# Autodesk Inventor assembly: s-assy-gripper
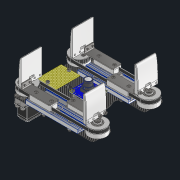
[picture p0: Inventor's stored thumbnail of the model, 180x180]
Saved by Autodesk Inventor 2021 (Build 250183000, 183)
## iProperties
Created: 2021-08-06
Part Number: s-assy-gripper
Document SubType Name: Assembly
Designer: yuta0
Mass: 588.108 g
Surface Area: 2137.5 cm^2
Volume: 253.038 cm^3
Density: 2.32419 g/cm^3
Author: yuta0
## Documents named in this file (25)
- C:\Users\yuta0\Documents\GitHub\catchrobo_hardware\assy-robot\s-assy-gripper.iam
- C:\Users\yuta0\Documents\GitHub\catchrobo_hardware\assy-robot\carbon_plate14.ipt
- C:\Users\yuta0\Documents\GitHub\catchrobo_hardware\assy-robot\mrs20-100.ipt
- C:\Users\yuta0\Documents\GitHub\catchrobo_hardware\assy-robot\mr-20cs_1.iam
- C:\Users\yuta0\Documents\GitHub\catchrobo_hardware\assy-robot\belt4.ipt
- C:\Users\yuta0\Documents\GitHub\catchrobo_hardware\assy-robot\base37.ipt
- C:\Users\yuta0\Documents\GitHub\catchrobo_hardware\assy-robot\USB Cam model ELP-USBFHD01M-L21.ipt
- C:\Users\yuta0\Documents\GitHub\catchrobo_hardware\assy-robot\CB3-5.ipt
- C:\Users\yuta0\Documents\GitHub\catchrobo_hardware\assy-robot\base38.ipt
- C:\Users\yuta0\Documents\GitHub\catchrobo_hardware\assy-robot\CB3-30.ipt
- C:\Users\yuta0\Documents\GitHub\catchrobo_hardware\assy-robot\LBNR4.ipt
- C:\Users\yuta0\Documents\GitHub\catchrobo_hardware\assy-robot\ARU-2010.ipt
- C:\Users\yuta0\Documents\GitHub\catchrobo_hardware\assy-robot\CB2-4.ipt
- C:\Users\yuta0\Documents\GitHub\catchrobo_hardware\assy-robot\d_type_board.ipt
- C:\Users\yuta0\Documents\GitHub\catchrobo_hardware\assy-robot\hexagonal_spacer_M3_5mm.ipt
- C:\Users\yuta0\Documents\GitHub\catchrobo_hardware\assy-robot\LBNR3.ipt
- C:\Users\yuta0\Documents\GitHub\catchrobo_hardware\assy-robot\steel_plate1.ipt
- C:\Users\yuta0\Documents\GitHub\catchrobo_hardware\assy-robot\CBSTNR3-16.ipt
- C:\Users\yuta0\Documents\GitHub\catchrobo_hardware\assy-robot\s-assy-rc_servo.iam
- C:\Users\yuta0\Documents\GitHub\catchrobo_hardware\assy-robot\s-assy-gripper_tentioner.iam
- C:\Users\yuta0\Documents\GitHub\catchrobo_hardware\assy-robot\FU650AD5-C6.ipt
- C:\Users\yuta0\Documents\GitHub\catchrobo_hardware\assy-robot\base21.ipt
- C:\Users\yuta0\Documents\GitHub\catchrobo_hardware\assy-robot\CBSTSR4-14.ipt
- C:\Users\yuta0\Documents\GitHub\catchrobo_hardware\assy-robot\base22.ipt
- C:\Users\yuta0\Documents\GitHub\catchrobo_hardware\assy-robot\CB3-10.ipt
## Components (93 placed, 24 different names)
1. carbon_plate14:1 — メイト:1, メイト:2, メイト:3, メイト:51, メイト:52, メイト:53, メイト:88, メイト:89, メイト:90, メイト:92, 角度:1, メイト:98, メイト:102, メイト:103, メイト:104, メイト:105, メイト:106, メイト:107, メイト:109, メイト:110, メイト:111, メイト:113, メイト:139, メイト:140, メイト:141, メイト:142, メイト:143, メイト:144, メイト:147, メイト:148, メイト:150, メイト:151, メイト:183, メイト:197, メイト:200, 角度:4, 角度:5, メイト:201, メイト:202, メイト:203, メイト:207, メイト:208
2. s-assy-rc_servo:1 [sub-assembly] — メイト:139, メイト:140, メイト:141, メイト:145, メイト:146
3. s-assy-rc_servo:2 [sub-assembly] — メイト:142, メイト:143, メイト:144, メイト:153, メイト:154
4. s-assy-gripper_tentioner:1 [sub-assembly] — メイト:147, メイト:148, メイト:149
5. s-assy-gripper_tentioner:2 [sub-assembly] — メイト:150, メイト:151, メイト:152
6. USB Cam model ELP-USBFHD01M-L21:1 — メイト:51, メイト:52, メイト:53, メイト:99, メイト:100, メイト:101
7. hexagonal_spacer_M3_5mm:1 — メイト:106, メイト:107, メイト:108, メイト:114
8. LBNR3:1 — メイト:108, メイト:109
9. LBNR3:2 — メイト:112, メイト:113
10. hexagonal_spacer_M3_5mm:2 — メイト:110, メイト:111, メイト:112
11. d_type_board:1 — メイト:104, メイト:105, メイト:114, メイト:115, メイト:116, メイト:117, メイト:118
12. CB3-5:11 — メイト:115, メイト:116
13. CB3-5:12 — メイト:117, メイト:118
14. belt4:1 — メイト:145, メイト:146, メイト:149
15. belt4:2 — メイト:152, メイト:153, メイト:154
16. FU650AD5-C6:1 — メイト:197, メイト:198, 角度:5
17. FU650AD5-C6:2 — メイト:199, メイト:200, 角度:4
18. base21:1 — メイト:201, メイト:202, メイト:203, メイト:204, メイト:205
19. base21:2 — メイト:206, メイト:207, メイト:208, メイト:209, メイト:210
20. CB3-30:1 — メイト:88, メイト:89
21. CB3-30:2
22. CB3-30:3
23. CB3-30:4
24. CB3-30:5
25. CB3-30:6
26. ARU-2010:1 — メイト:98, メイト:99
27. CB2-4:1 — メイト:100, メイト:101
28. CB2-4:2 — メイト:102, メイト:103
29. ARU-2010:2
30. CB2-4:3
31. CB2-4:6
32. ARU-2010:3
33. CB2-4:4
34. CB2-4:7
35. ARU-2010:4
36. CB2-4:5
37. CB2-4:8
38. CBSTNR3-16:4 — メイト:194, メイト:211
39. CBSTNR3-16:3 — メイト:193
40. steel_plate1:2 — メイト:195, メイト:196, メイト:212, メイト:213, メイト:214
41. base38:2 — メイト:195, メイト:196
42. base37:2 — メイト:211
43. mr-20cs_1:2 [sub-assembly] — メイト:193, メイト:194
44. CBSTSR4-14:1
45. LBNR4:4 — メイト:204
46. CBSTSR4-14:2
47. LBNR4:3 — メイト:205
48. base22:1 — メイト:212, メイト:213, メイト:214, メイト:215, メイト:216, メイト:217, メイト:218
49. CB3-10:1 — メイト:215, メイト:216
50. CB3-10:2 — メイト:217, メイト:218
51. mrs20-100:2 — メイト:183, メイト:198
52. CBSTNR3-16:5
53. CBSTNR3-16:6
54. steel_plate1:3
55. base38:3
56. base37:3
57. mr-20cs_1:3 [sub-assembly]
58. CBSTSR4-14:5
59. LBNR4:5
60. CBSTSR4-14:6
61. LBNR4:6
62. base22:3
63. CB3-10:5
64. CB3-10:6
65. mrs20-100:3
66. steel_plate1:1 — メイト:129, メイト:130, メイト:131, メイト:133, メイト:134, メイト:135, メイト:219, メイト:220, メイト:221
67. CBSTNR3-16:1 — メイト:132, メイト:133
68. CBSTNR3-16:2 — メイト:134, メイト:135
69. base37:1 — メイト:45, メイト:46, メイト:47, メイト:70, メイト:71, メイト:72
70. base38:1 — メイト:70, メイト:71, メイト:72, メイト:129, メイト:130, メイト:131, メイト:132
71. mr-20cs_1:1 [sub-assembly] — メイト:7, メイト:8, フラッシュ:1, メイト:45, メイト:46, メイト:47
72. mrs20-100:1 — フラッシュ:1, メイト:1, メイト:2, メイト:3, メイト:7, メイト:8, メイト:199
73. CBSTSR4-14:3
74. LBNR4:1 — メイト:90, 角度:2, メイト:210
75. CBSTSR4-14:4 — メイト:206
76. LBNR4:2 — メイト:92, 角度:1, 角度:2, メイト:209
77. CB3-10:4 — メイト:223
78. CB3-10:3 — メイト:222
79. base22:2 — メイト:219, メイト:220, メイト:221, メイト:222, メイト:223
80. steel_plate1:4
81. CBSTNR3-16:7
82. CBSTNR3-16:8
83. base37:4
84. base38:4
85. mr-20cs_1:4 [sub-assembly]
86. mrs20-100:4
87. CBSTSR4-14:7
88. LBNR4:7
89. CBSTSR4-14:8
90. LBNR4:8
91. CB3-10:7
92. CB3-10:8
93. base22:4
## Component patterns: (6 elements, first: CB3-30:1), (4 elements, first: ARU-2010:1 + CB2-4:1 + CB2-4:2), (2 elements, first: CBSTNR3-16:4 + CBSTNR3-16:3 + steel_plate1:2 + base38:2 + base37:2 + mr-20cs_1:2 + CBSTSR4-14:1 + LBNR4:4 + CBSTSR4-14:2 + LBNR4:3 + base22:1 + CB3-10:1 + CB3-10:2 + mrs20-100:2), (2 elements, first: steel_plate1:1 + CBSTNR3-16:1 + CBSTNR3-16:2 + base37:1 + base38:1 + mr-20cs_1:1 + mrs20-100:1 + CBSTSR4-14:3 + LBNR4:1 + CBSTSR4-14:4 + LBNR4:2 + CB3-10:4 + CB3-10:3 + base22:2)
## Relationships (125: Mate 118, Angle 5, Flush 2)
- フラッシュ:1 [Flush]: mr-20cs_1:1 ↔ mrs20-100:1
- メイト:1 [Mate]: carbon_plate14:1 ↔ mrs20-100:1
- メイト:2 [Mate]: carbon_plate14:1 ↔ mrs20-100:1
- メイト:3 [Mate]: carbon_plate14:1 ↔ mrs20-100:1
- メイト:7 [Mate] (0.1 mm): mr-20cs_1:1 ↔ mrs20-100:1
- メイト:8 [Mate] (0.15 mm): mr-20cs_1:1 ↔ mrs20-100:1
- メイト:45 [Mate]: base37:1 ↔ mr-20cs_1:1
- メイト:46 [Mate]: base37:1 ↔ mr-20cs_1:1
- メイト:47 [Mate]: base37:1 ↔ mr-20cs_1:1
- メイト:51 [Mate] (10 mm): carbon_plate14:1 ↔ USB Cam model ELP-USBFHD01M-L21:1
- メイト:52 [Mate]: carbon_plate14:1 ↔ USB Cam model ELP-USBFHD01M-L21:1
- メイト:53 [Mate]: carbon_plate14:1 ↔ USB Cam model ELP-USBFHD01M-L21:1
- メイト:70 [Mate]: base37:1 ↔ base38:1
- メイト:71 [Mate]: base37:1 ↔ base38:1
- メイト:72 [Mate]: base37:1 ↔ base38:1
- メイト:88 [Mate]: carbon_plate14:1 ↔ CB3-30:1
- メイト:89 [Mate]: carbon_plate14:1 ↔ CB3-30:1
- メイト:90 [Mate]: carbon_plate14:1 ↔ LBNR4:1
- メイト:92 [Mate]: carbon_plate14:1 ↔ LBNR4:2
- 角度:1 [Angle] (0 deg): carbon_plate14:1 ↔ LBNR4:2
- 角度:2 [Angle] (0 deg): LBNR4:1 ↔ LBNR4:2
- メイト:98 [Mate]: carbon_plate14:1 ↔ ARU-2010:1
- メイト:99 [Mate]: USB Cam model ELP-USBFHD01M-L21:1 ↔ ARU-2010:1
- メイト:100 [Mate]: USB Cam model ELP-USBFHD01M-L21:1 ↔ CB2-4:1
- メイト:101 [Mate]: USB Cam model ELP-USBFHD01M-L21:1 ↔ CB2-4:1
- メイト:102 [Mate]: carbon_plate14:1 ↔ CB2-4:2
- メイト:103 [Mate]: carbon_plate14:1 ↔ CB2-4:2
- メイト:104 [Mate]: carbon_plate14:1 ↔ d_type_board:1
- メイト:105 [Mate]: carbon_plate14:1 ↔ d_type_board:1
- メイト:106 [Mate]: carbon_plate14:1 ↔ hexagonal_spacer_M3_5mm:1
- メイト:107 [Mate]: carbon_plate14:1 ↔ hexagonal_spacer_M3_5mm:1
- メイト:108 [Mate]: hexagonal_spacer_M3_5mm:1 ↔ LBNR3:1
- メイト:109 [Mate]: carbon_plate14:1 ↔ LBNR3:1
- メイト:110 [Mate]: carbon_plate14:1 ↔ hexagonal_spacer_M3_5mm:2
- メイト:111 [Mate]: carbon_plate14:1 ↔ hexagonal_spacer_M3_5mm:2
- メイト:112 [Mate]: LBNR3:2 ↔ hexagonal_spacer_M3_5mm:2
- メイト:113 [Mate]: carbon_plate14:1 ↔ LBNR3:2
- メイト:114 [Mate]: hexagonal_spacer_M3_5mm:1 ↔ d_type_board:1
- メイト:115 [Mate]: d_type_board:1 ↔ CB3-5:11
- メイト:116 [Mate]: d_type_board:1 ↔ CB3-5:11
- メイト:117 [Mate]: d_type_board:1 ↔ CB3-5:12
- メイト:118 [Mate]: d_type_board:1 ↔ CB3-5:12
- [Mate]: mrs20-100:1 ↔ CBSTSR4-14:3
- [Mate]: mrs20-100:1 ↔ CBSTSR4-14:3
- [Mate]: mrs20-100:1 ↔ CBSTSR4-14:4
- [Mate]: mrs20-100:1 ↔ CBSTSR4-14:4
- メイト:129 [Mate]: steel_plate1:1 ↔ base38:1
- メイト:130 [Mate]: steel_plate1:1 ↔ base38:1
- メイト:131 [Mate]: steel_plate1:1 ↔ base38:1
- メイト:132 [Mate]: CBSTNR3-16:1 ↔ base38:1
- メイト:133 [Mate]: steel_plate1:1 ↔ CBSTNR3-16:1
- メイト:134 [Mate]: steel_plate1:1 ↔ CBSTNR3-16:2
- メイト:135 [Mate]: steel_plate1:1 ↔ CBSTNR3-16:2
- [Mate]: steel_plate1:1 ↔ CB3-10:4
- [Mate]: steel_plate1:1 ↔ CB3-10:3
- メイト:139 [Mate]: carbon_plate14:1 ↔ s-assy-rc_servo:1
- メイト:140 [Mate]: carbon_plate14:1 ↔ s-assy-rc_servo:1
- メイト:141 [Mate]: carbon_plate14:1 ↔ s-assy-rc_servo:1
- メイト:142 [Mate]: carbon_plate14:1 ↔ s-assy-rc_servo:2
- メイト:143 [Mate]: carbon_plate14:1 ↔ s-assy-rc_servo:2
- メイト:144 [Mate]: carbon_plate14:1 ↔ s-assy-rc_servo:2
- メイト:145 [Mate]: s-assy-rc_servo:1 ↔ belt4:1
- メイト:146 [Mate] (0.5 mm): s-assy-rc_servo:1 ↔ belt4:1
- メイト:147 [Mate]: carbon_plate14:1 ↔ s-assy-gripper_tentioner:1
- メイト:148 [Mate]: carbon_plate14:1 ↔ s-assy-gripper_tentioner:1
- メイト:149 [Mate]: s-assy-gripper_tentioner:1 ↔ belt4:1
- メイト:150 [Mate]: carbon_plate14:1 ↔ s-assy-gripper_tentioner:2
- メイト:151 [Mate]: carbon_plate14:1 ↔ s-assy-gripper_tentioner:2
- メイト:152 [Mate]: s-assy-gripper_tentioner:2 ↔ belt4:2
- メイト:153 [Mate]: s-assy-rc_servo:2 ↔ belt4:2
- メイト:154 [Mate] (0.5 mm): s-assy-rc_servo:2 ↔ belt4:2
- [Flush]: mr-20cs_1:2 ↔ mrs20-100:2
- [Mate] (0.1 mm): mr-20cs_1:2 ↔ mrs20-100:2
- [Mate] (0.15 mm): mr-20cs_1:2 ↔ mrs20-100:2
- [Mate]: base37:2 ↔ mr-20cs_1:2
- [Mate]: base38:2 ↔ base37:2
- [Mate]: base38:2 ↔ base37:2
- [Mate]: base38:2 ↔ base37:2
- [Angle] (0 deg): LBNR4:4 ↔ LBNR4:3
- [Mate]: CBSTSR4-14:2 ↔ mrs20-100:2
- [Mate]: CBSTSR4-14:2 ↔ mrs20-100:2
- [Mate]: CBSTSR4-14:1 ↔ mrs20-100:2
- [Mate]: CBSTSR4-14:1 ↔ mrs20-100:2
- [Mate]: steel_plate1:2 ↔ base38:2
- [Mate]: CBSTNR3-16:3 ↔ base38:2
- [Mate]: CBSTNR3-16:3 ↔ steel_plate1:2
- [Mate]: CBSTNR3-16:4 ↔ steel_plate1:2
- [Mate]: carbon_plate14:1 ↔ CBSTSR4-14:2
- [Mate]: carbon_plate14:1 ↔ CBSTSR4-14:1
- メイト:183 [Mate]: carbon_plate14:1 ↔ mrs20-100:2
- [Mate]: CBSTSR4-14:1 ↔ LBNR4:4
- [Mate]: CBSTSR4-14:2 ↔ LBNR4:3
- メイト:193 [Mate]: CBSTNR3-16:3 ↔ mr-20cs_1:2
- メイト:194 [Mate]: CBSTNR3-16:4 ↔ mr-20cs_1:2
- メイト:195 [Mate]: steel_plate1:2 ↔ base38:2
- メイト:196 [Mate]: steel_plate1:2 ↔ base38:2
- メイト:197 [Mate]: carbon_plate14:1 ↔ FU650AD5-C6:1
- メイト:198 [Mate]: FU650AD5-C6:1 ↔ mrs20-100:2
- メイト:199 [Mate]: FU650AD5-C6:2 ↔ mrs20-100:1
- メイト:200 [Mate]: carbon_plate14:1 ↔ FU650AD5-C6:2
- 角度:4 [Angle] (0 deg): carbon_plate14:1 ↔ FU650AD5-C6:2
- 角度:5 [Angle] (0 deg): carbon_plate14:1 ↔ FU650AD5-C6:1
- メイト:201 [Mate]: carbon_plate14:1 ↔ base21:1
- メイト:202 [Mate]: carbon_plate14:1 ↔ base21:1
- メイト:203 [Mate]: carbon_plate14:1 ↔ base21:1
- メイト:204 [Mate]: base21:1 ↔ LBNR4:4
- メイト:205 [Mate]: base21:1 ↔ LBNR4:3
- メイト:206 [Mate]: base21:2 ↔ CBSTSR4-14:4
- メイト:207 [Mate]: carbon_plate14:1 ↔ base21:2
- メイト:208 [Mate]: carbon_plate14:1 ↔ base21:2
- メイト:209 [Mate]: base21:2 ↔ LBNR4:2
- メイト:210 [Mate]: base21:2 ↔ LBNR4:1
- メイト:211 [Mate]: CBSTNR3-16:4 ↔ base37:2
- メイト:212 [Mate]: steel_plate1:2 ↔ base22:1
- メイト:213 [Mate]: steel_plate1:2 ↔ base22:1
- メイト:214 [Mate]: steel_plate1:2 ↔ base22:1
- メイト:215 [Mate]: base22:1 ↔ CB3-10:1
- メイト:216 [Mate]: base22:1 ↔ CB3-10:1
- メイト:217 [Mate]: base22:1 ↔ CB3-10:2
- メイト:218 [Mate]: base22:1 ↔ CB3-10:2
- メイト:219 [Mate]: steel_plate1:1 ↔ base22:2
- メイト:220 [Mate]: steel_plate1:1 ↔ base22:2
- メイト:221 [Mate]: steel_plate1:1 ↔ base22:2
- メイト:222 [Mate]: CB3-10:3 ↔ base22:2
- メイト:223 [Mate]: CB3-10:4 ↔ base22:2
## Named parameters: d270_d237 = 0 mm, d271_d238 = 0 mm, d273_d240 = 0 mm, d279_d230 = 0 mm, d280_d22 = 0.1 mm, d281_d23 = 0.15 mm, d282_d214 = 0 mm, d283_d215 = 0 mm, d284_d216 = 0 mm, d285_d217 = 0 mm, d286_d170 = 0 deg, d289_d106 = 0 mm, d294_d139 = 0 mm, d295_d140 = 0 mm, d296_d141 = 0 mm, d297_d26 = 0 mm
